# Autodesk Inventor assembly: 6060gantry
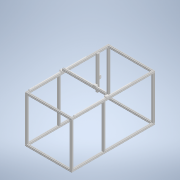
[picture p0: Inventor's stored thumbnail of the model, 180x180]
Saved by Autodesk Inventor 2022 (Build 260153000, 153)
## iProperties
Created: 2021-06-21
Part Number: 6060gantry
Document SubType Name: Assembly
Designer: lyndsaygreen
Author: lyndsaygreen
## Documents named in this file (7)
- \\Mac\Home\Desktop\WinnipegPMTTestFacility\gantry design\6060gantry.iam
- \\Mac\Home\Desktop\WinnipegPMTTestFacility\gantry design\GFS8-6060-1000_Autodesk_Inventor_2020_20210621\GFS8-6060-1000.ipt
- \\Mac\Home\Desktop\WinnipegPMTTestFacility\gantry design\GFS8-6060-1000_Autodesk_Inventor_2020_20210621\6060-5.5.ipt
- \\Mac\Home\Desktop\WinnipegPMTTestFacility\gantry design\GFS8-6060-1000_Autodesk_Inventor_2020_20210621\6060-3.5.ipt
- \\Mac\Home\Desktop\WinnipegPMTTestFacility\gantry design\THK_HSR35R1SS280LG200BM6F8530001R2\AIS2020\HSR35R1SS-280L_G20_0_B-M6F_85-3_0_0_0_1_(R2).iam
- \\Mac\Home\Desktop\WinnipegPMTTestFacility\gantry design\THK_HSR35R1SS280LG200BM6F8530001R20\AIS2020\HSR35R1SS-280L_G20_0_B-M6F_85-3_0_0_0_1_(R2).iam
- \\Mac\Home\Desktop\WinnipegPMTTestFacility\gantry design\THK_HSR35R1SS280LG200BM6F8530001R2-2\AIS2020\HSR35R1SS-280L_G20_0_B-M6F_85-3_0_0_0_1_(R2).iam
## Components (20 placed, 4 different names)
1. GFS8-6060-1000:2 — Mate:1, Flush:1, Flush:2, Mate:3, Mate:6, Flush:11, Flush:12, Mate:7, Flush:13, Flush:14, Mate:14, Flush:24, Mate:26
2. GFS8-6060-1000:3 — Mate:17, Flush:29, Flush:30, Mate:18, Flush:31, Flush:32, Mate:21, Flush:36, Flush:37
3. GFS8-6060-1000:5 — Mate:2, Flush:3, Flush:4, Flush:5, Flush:6, Mate:4, Flush:7, Flush:8, Mate:5, Flush:9, Flush:10, Mate:13, Flush:23
4. GFS8-6060-1000:6 — Mate:15, Flush:25, Flush:26, Mate:16, Flush:27, Mate:20, Flush:34, Flush:35
5. 6060-5.5:1 — Mate:7, Flush:13, Flush:14, Flush:26, Mate:17, Flush:29, Flush:30
6. 6060-5.5:2 — Mate:13, Flush:23, Flush:33
7. 6060-5.5:3 — Mate:6, Flush:11, Flush:12, Mate:19
8. 6060-5.5:4 — Mate:14, Flush:24, Mate:19, Flush:33
9. 6060-5.5:5 — Mate:5, Flush:9, Flush:10
10. 6060-5.5:6 — Mate:4, Flush:7, Flush:8, Mate:15, Flush:25, Flush:28
11. 6060-5.5:7 — Mate:16, Flush:27, Flush:28
12. 6060-5.5:8 — Mate:3, Flush:5, Flush:6
13. 6060-5.5:9 — Mate:1, Flush:1, Flush:2, Mate:2, Flush:3, Flush:4
14. 6060-5.5:10 — Mate:18, Flush:31, Flush:32
15. 6060-5.5:11 — Flush:38, Mate:22, Mate:23, Mate:24, Flush:40, Flush:43
16. 6060-3.5:1 — Mate:25, Flush:41, Mate:26, Mate:27, Flush:42, Flush:44
17. HSR35R1SS-280L_G20_0_B-M6F_85-3_0_0_0_1_(R2):1 [sub-assembly] — Mate:21, Flush:36, Flush:37, Flush:38, Mate:22, Mate:23
18. HSR35R1SS-280L_G20_0_B-M6F_85-3_0_0_0_1_(R2):2 [sub-assembly] — Mate:20, Flush:34, Flush:35
19. HSR35R1SS-280L_G20_0_B-M6F_85-3_0_0_0_1_(R2):3 [sub-assembly] — Mate:24, Flush:40, Mate:25, Flush:41, Flush:43
20. HSR35R1SS-280L_G20_0_B-M6F_85-3_0_0_0_1_(R2):5 [sub-assembly] — Mate:27, Flush:42, Flush:44
## Relationships (57: Flush 35, Mate 22)
- Mate:1: GFS8-6060-1000:2 ↔ 6060-5.5:9
- Flush:1: GFS8-6060-1000:2 ↔ 6060-5.5:9
- Flush:2: GFS8-6060-1000:2 ↔ 6060-5.5:9
- Mate:2: GFS8-6060-1000:5 ↔ 6060-5.5:9
- Flush:3: GFS8-6060-1000:5 ↔ 6060-5.5:9
- Flush:4: GFS8-6060-1000:5 ↔ 6060-5.5:9
- Mate:3: GFS8-6060-1000:2 ↔ 6060-5.5:8
- Flush:5: GFS8-6060-1000:5 ↔ 6060-5.5:8
- Flush:6: GFS8-6060-1000:5 ↔ 6060-5.5:8
- Mate:4: GFS8-6060-1000:5 ↔ 6060-5.5:6
- Flush:7: GFS8-6060-1000:5 ↔ 6060-5.5:6
- Flush:8: GFS8-6060-1000:5 ↔ 6060-5.5:6
- Mate:5: GFS8-6060-1000:5 ↔ 6060-5.5:5
- Flush:9: GFS8-6060-1000:5 ↔ 6060-5.5:5
- Flush:10: GFS8-6060-1000:5 ↔ 6060-5.5:5
- Mate:6: GFS8-6060-1000:2 ↔ 6060-5.5:3
- Flush:11: GFS8-6060-1000:2 ↔ 6060-5.5:3
- Flush:12: GFS8-6060-1000:2 ↔ 6060-5.5:3
- Mate:7: GFS8-6060-1000:2 ↔ 6060-5.5:1
- Flush:13: GFS8-6060-1000:2 ↔ 6060-5.5:1
- Flush:14: GFS8-6060-1000:2 ↔ 6060-5.5:1
- Mate:13: GFS8-6060-1000:5 ↔ 6060-5.5:2
- Flush:23: GFS8-6060-1000:5 ↔ 6060-5.5:2
- Mate:14: GFS8-6060-1000:2 ↔ 6060-5.5:4
- Flush:24: GFS8-6060-1000:2 ↔ 6060-5.5:4
- Mate:15: GFS8-6060-1000:6 ↔ 6060-5.5:6
- Flush:25: GFS8-6060-1000:6 ↔ 6060-5.5:6
- Flush:26: GFS8-6060-1000:6 ↔ 6060-5.5:1
- Mate:16: GFS8-6060-1000:6 ↔ 6060-5.5:7
- Flush:27: GFS8-6060-1000:6 ↔ 6060-5.5:7
- Flush:28: 6060-5.5:6 ↔ 6060-5.5:7
- Mate:17: GFS8-6060-1000:3 ↔ 6060-5.5:1
- Flush:29: GFS8-6060-1000:3 ↔ 6060-5.5:1
- Flush:30: GFS8-6060-1000:3 ↔ 6060-5.5:1
- Mate:18: GFS8-6060-1000:3 ↔ 6060-5.5:10
- Flush:31: GFS8-6060-1000:3 ↔ 6060-5.5:10
- Flush:32: GFS8-6060-1000:3 ↔ 6060-5.5:10
- Mate:19 (1524 mm): 6060-5.5:3 ↔ 6060-5.5:4
- Flush:33: 6060-5.5:2 ↔ 6060-5.5:4
- Mate:20: GFS8-6060-1000:6 ↔ HSR35R1SS-280L_G20_0_B-M6F_85-3_0_0_0_1_(R2):2
- Flush:34 (-101.6 mm): GFS8-6060-1000:6 ↔ HSR35R1SS-280L_G20_0_B-M6F_85-3_0_0_0_1_(R2):2
- Flush:35 (-13.208 mm): GFS8-6060-1000:6 ↔ HSR35R1SS-280L_G20_0_B-M6F_85-3_0_0_0_1_(R2):2
- Mate:21: GFS8-6060-1000:3 ↔ HSR35R1SS-280L_G20_0_B-M6F_85-3_0_0_0_1_(R2):1
- Flush:36 (101.6 mm): GFS8-6060-1000:3 ↔ HSR35R1SS-280L_G20_0_B-M6F_85-3_0_0_0_1_(R2):1
- Flush:37 (-13.208 mm): GFS8-6060-1000:3 ↔ HSR35R1SS-280L_G20_0_B-M6F_85-3_0_0_0_1_(R2):1
- Flush:38 (10.16 mm): 6060-5.5:11 ↔ HSR35R1SS-280L_G20_0_B-M6F_85-3_0_0_0_1_(R2):1
- Mate:22: 6060-5.5:11 ↔ HSR35R1SS-280L_G20_0_B-M6F_85-3_0_0_0_1_(R2):1
- Mate:23 (-6.35 mm): 6060-5.5:11 ↔ HSR35R1SS-280L_G20_0_B-M6F_85-3_0_0_0_1_(R2):1
- Mate:24: 6060-5.5:11 ↔ HSR35R1SS-280L_G20_0_B-M6F_85-3_0_0_0_1_(R2):3
- Flush:40 (-12.7 mm): 6060-5.5:11 ↔ HSR35R1SS-280L_G20_0_B-M6F_85-3_0_0_0_1_(R2):3
- Mate:25: 6060-3.5:1 ↔ HSR35R1SS-280L_G20_0_B-M6F_85-3_0_0_0_1_(R2):3
- Flush:41 (-8.89 mm): 6060-3.5:1 ↔ HSR35R1SS-280L_G20_0_B-M6F_85-3_0_0_0_1_(R2):3
- Mate:26 (1371.6 mm): GFS8-6060-1000:2 ↔ 6060-3.5:1
- Mate:27: 6060-3.5:1 ↔ HSR35R1SS-280L_G20_0_B-M6F_85-3_0_0_0_1_(R2):5
- Flush:42: 6060-3.5:1 ↔ HSR35R1SS-280L_G20_0_B-M6F_85-3_0_0_0_1_(R2):5
- Flush:43: 6060-5.5:11 ↔ HSR35R1SS-280L_G20_0_B-M6F_85-3_0_0_0_1_(R2):3
- Flush:44 (12.7 mm): 6060-3.5:1 ↔ HSR35R1SS-280L_G20_0_B-M6F_85-3_0_0_0_1_(R2):5
